# Autodesk Inventor assembly: batterieEtCacheBatterie
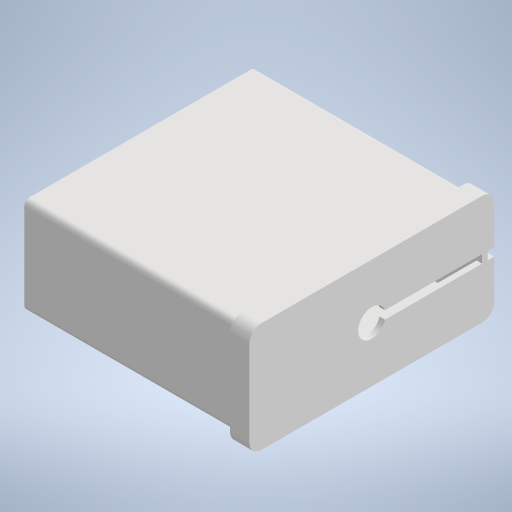
[picture p0: Inventor's stored thumbnail of the model, 512x512]
Saved by Autodesk Inventor 2023 (Build 270158000, 158)
## iProperties
Created: 2023-03-28
Part Number: batterieEtCacheBatterie
Document SubType Name: Assembly
Designer: eleves
Author: eleves
## Documents named in this file (3)
- C:\Users\eleves\Desktop\PE-SM\3D\batterieEtCacheBatterie.iam
- C:\Users\eleves\Desktop\PE-SM\3D\BatterieHolder.ipt
- C:\Users\eleves\Desktop\PE-SM\3D\cache_batterie_1.ipt
## Components (2 placed, 2 different names)
1. BatterieHolder:1 — Affleurement:1, Affleurement:2
2. cache_batterie_1:1 — Affleurement:1, Affleurement:2
## Relationships (2: Flush 2)
- Affleurement:1 [Flush]: BatterieHolder:1 ↔ cache_batterie_1:1
- Affleurement:2 [Flush]: BatterieHolder:1 ↔ cache_batterie_1:1
